# Autodesk Inventor assembly: Bumpers
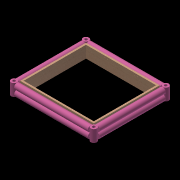
[picture p0: Inventor's stored thumbnail of the model, 180x180]
Saved by Autodesk Inventor 2014 SP1 (Build 180222100, 222)
## iProperties
Created: 2013-11-29
Part Number: Bumpers
Document SubType Name: Assembly
Designer: Rauhul Varma
Author: Rauhul Varma
## Documents named in this file (6)
- C:\Users\Rauhul Varma\Desktop\2014 Base\Bumpers.iam
- C:\Users\Rauhul Varma\Desktop\2014 Base\Bumper Wood Front.ipt
- C:\Users\Rauhul Varma\Desktop\2014 Base\Bumper Wood Side.ipt
- C:\Users\Rauhul Varma\Desktop\2014 Base\Pool Noodle Front.ipt
- C:\Users\Rauhul Varma\Desktop\2014 Base\Pool Noodle Side.ipt
- C:\Users\Rauhul Varma\Desktop\2014 Base\Pool Noodle Vertical.ipt
## Components (16 placed, 5 different names)
1. Bumper Wood Front:1 — Mate:1, Flush:1, Flush:2, Mate:2, Flush:3, Flush:4, Tangent:17, Tangent:18, Tangent:19, Tangent:20
2. Bumper Wood Side:1 — Mate:1, Flush:1, Flush:2, Mate:3, Flush:5, Flush:6, Tangent:5, Tangent:6, Tangent:7, Tangent:8, Flush:9, Flush:10, Flush:11, Flush:12, Flush:15, Flush:16, Flush:18
3. Bumper Wood Front:2 — Mate:3, Flush:5, Flush:6, Tangent:9, Tangent:10, Tangent:11, Tangent:12, Flush:13, Flush:14
4. Bumper Wood Side:2 — Mate:2, Flush:3, Flush:4, Tangent:1, Tangent:2, Flush:7, Tangent:3, Tangent:4, Flush:8, Flush:17
5. Pool Noodle Front:1 — Tangent:9, Tangent:12, Flush:11
6. Pool Noodle Side:1 — Tangent:1, Tangent:2, Flush:7, Tangent:15, Tangent:23
7. Pool Noodle Vertical:1 — Tangent:15, Tangent:16, Flush:14
8. Pool Noodle Side:2 — Tangent:5, Tangent:7, Flush:10, Tangent:13, Tangent:22
9. Pool Noodle Side:3 — Tangent:3, Tangent:4, Flush:8
10. Pool Noodle Side:4 — Tangent:6, Tangent:8, Flush:9
11. Pool Noodle Front:2 — Tangent:18, Tangent:20, Flush:15
12. Pool Noodle Front:3 — Tangent:10, Tangent:11, Flush:12, Tangent:14, Tangent:16
13. Pool Noodle Front:4 — Tangent:17, Tangent:19, Flush:16, Tangent:21, Tangent:24
14. Pool Noodle Vertical:2 — Tangent:21, Tangent:22, Flush:18
15. Pool Noodle Vertical:3 — Tangent:23, Tangent:24, Flush:17
16. Pool Noodle Vertical:4 — Tangent:13, Tangent:14, Flush:13
## Relationships (45: Tangent 24, Flush 18, Mate 3)
- Mate:1: Bumper Wood Front:1 ↔ Bumper Wood Side:1
- Flush:1: Bumper Wood Front:1 ↔ Bumper Wood Side:1
- Flush:2: Bumper Wood Front:1 ↔ Bumper Wood Side:1
- Mate:2: Bumper Wood Front:1 ↔ Bumper Wood Side:2
- Flush:3: Bumper Wood Front:1 ↔ Bumper Wood Side:2
- Flush:4: Bumper Wood Front:1 ↔ Bumper Wood Side:2
- Mate:3: Bumper Wood Side:1 ↔ Bumper Wood Front:2
- Flush:5: Bumper Wood Side:1 ↔ Bumper Wood Front:2
- Flush:6: Bumper Wood Side:1 ↔ Bumper Wood Front:2
- Tangent:1: Bumper Wood Side:2 ↔ Pool Noodle Side:1
- Tangent:2: Bumper Wood Side:2 ↔ Pool Noodle Side:1
- Flush:7: Bumper Wood Side:2 ↔ Pool Noodle Side:1
- Tangent:3: Bumper Wood Side:2 ↔ Pool Noodle Side:3
- Tangent:4: Bumper Wood Side:2 ↔ Pool Noodle Side:3
- Flush:8: Bumper Wood Side:2 ↔ Pool Noodle Side:3
- Tangent:5: Bumper Wood Side:1 ↔ Pool Noodle Side:2
- Tangent:6: Bumper Wood Side:1 ↔ Pool Noodle Side:4
- Tangent:7: Bumper Wood Side:1 ↔ Pool Noodle Side:2
- Tangent:8: Bumper Wood Side:1 ↔ Pool Noodle Side:4
- Flush:9: Bumper Wood Side:1 ↔ Pool Noodle Side:4
- Flush:10: Bumper Wood Side:1 ↔ Pool Noodle Side:2
- Tangent:9: Bumper Wood Front:2 ↔ Pool Noodle Front:1
- Tangent:10: Bumper Wood Front:2 ↔ Pool Noodle Front:3
- Tangent:11: Bumper Wood Front:2 ↔ Pool Noodle Front:3
- Tangent:12: Bumper Wood Front:2 ↔ Pool Noodle Front:1
- Flush:11: Bumper Wood Side:1 ↔ Pool Noodle Front:1
- Flush:12: Bumper Wood Side:1 ↔ Pool Noodle Front:3
- Tangent:13: Pool Noodle Side:2 ↔ Pool Noodle Vertical:4
- Tangent:14: Pool Noodle Front:3 ↔ Pool Noodle Vertical:4
- Flush:13: Bumper Wood Front:2 ↔ Pool Noodle Vertical:4
- Tangent:15: Pool Noodle Side:1 ↔ Pool Noodle Vertical:1
- Tangent:16: Pool Noodle Vertical:1 ↔ Pool Noodle Front:3
- Flush:14: Bumper Wood Front:2 ↔ Pool Noodle Vertical:1
- Tangent:17: Bumper Wood Front:1 ↔ Pool Noodle Front:4
- Tangent:18: Bumper Wood Front:1 ↔ Pool Noodle Front:2
- Tangent:19: Bumper Wood Front:1 ↔ Pool Noodle Front:4
- Tangent:20: Bumper Wood Front:1 ↔ Pool Noodle Front:2
- Flush:15: Bumper Wood Side:1 ↔ Pool Noodle Front:2
- Flush:16: Bumper Wood Side:1 ↔ Pool Noodle Front:4
- Tangent:21: Pool Noodle Front:4 ↔ Pool Noodle Vertical:2
- Tangent:22: Pool Noodle Side:2 ↔ Pool Noodle Vertical:2
- Tangent:23: Pool Noodle Side:1 ↔ Pool Noodle Vertical:3
- Tangent:24: Pool Noodle Front:4 ↔ Pool Noodle Vertical:3
- Flush:17: Bumper Wood Side:2 ↔ Pool Noodle Vertical:3
- Flush:18: Bumper Wood Side:1 ↔ Pool Noodle Vertical:2
